# Autodesk Inventor assembly: Attempt 2
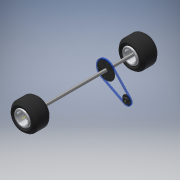
[picture p0: Inventor's stored thumbnail of the model, 180x180]
Saved by Autodesk Inventor 2016 (Build 200138000, 138)
## iProperties
Created: 2015-06-01
Part Number: Attempt 2
Document SubType Name: Assembly
Designer: Dennis
Mass: 27232.7 g
Surface Area: 12496.7 cm^2
Volume: 17666.9 cm^3
Density: 1.54146 g/cm^3
Author: Dennis
## Documents named in this file (4)
- C:\Users\jonathan\Desktop\CLEAN COPIES\GoCart Transmission\Inventor\Assembly.iam
- C:\Users\jonathan\Desktop\CLEAN COPIES\GoCart Transmission\Inventor\Driving Sprocket.ipt
- C:\Users\jonathan\Desktop\CLEAN COPIES\GoCart Transmission\Inventor\Chain Drive.iam
- C:\Users\jonathan\Desktop\CLEAN COPIES\GoCart Transmission\Inventor\Sprocket Axle and Wheel.iam
## Components (3 placed, 3 different names)
1. Chain Drive:1 [sub-assembly] — Mate:6, Mate:9
2. Sprocket Axle and Wheel:1 [sub-assembly] — Mate:6, Mate:7, Rotation:1
3. Driving Sprocket:1 — Mate:8, Mate:9, Rotation:1
## Relationships (5: Mate 4, RelateRotation 1)
- Mate:6: Chain Drive:1 ↔ Sprocket Axle and Wheel:1
- Mate:7: Sprocket Axle and Wheel:1
- Mate:8: Driving Sprocket:1
- Mate:9: Chain Drive:1 ↔ Driving Sprocket:1
- Rotation:1 [RelateRotation] (0.5 ul): Sprocket Axle and Wheel:1 ↔ Driving Sprocket:1
